# Autodesk Inventor assembly: Gearbox2F
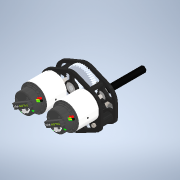
[picture p0: Inventor's stored thumbnail of the model, 180x180]
Saved by Autodesk Inventor 2022 (Build 260153000, 153)
## iProperties
Created: 2022-01-10
Part Number: Gearbox2F
Document SubType Name: Assembly
Designer: merky
Author: merky
## Documents named in this file (7)
- C:\Users\Daniel Marquez\Documents\t3-cad\CAD\2022 Parts\Generic\Gearbox2F.iam
- C:\Users\Daniel Marquez\Documents\t3-cad\CAD\WCP SS_Shrinkwrap.ipt
- C:\Users\Daniel Marquez\Documents\t3-cad\CAD\2022 Parts\Generic\Falcon500.ipt
- C:\Users\Daniel Marquez\Documents\t3-cad\CAD\WCP DS Gearbox\217-2734.ipt
- C:\Users\Daniel Marquez\Documents\t3-cad\CAD\WCP DS Gearbox\217-3422-007 Rev1.ipt
- C:\Users\Daniel Marquez\Documents\t3-cad\CAD\WCP DS Gearbox\217-3422-004 Rev2.ipt
- C:\Users\Daniel Marquez\Documents\t3-cad\CAD\2022 Parts\Generic\9inthundershaft.ipt
## Components (8 placed, 6 different names)
1. WCP SS_Shrinkwrap:1 — Insert:1, Insert:2, Insert:5
2. Falcon500:1 — Insert:2
3. Falcon500:2 — Insert:1
4. 217-2734:1 — Mate:5, Mate:6
5. 217-3422-007 Rev1:1 — Insert:4
6. 217-3422-007 Rev1:2 — Insert:3
7. 217-3422-004 Rev2:1 — Insert:3, Insert:4, Insert:5
8. 9inthundershaft:1 — Mate:5, Mate:6
## Relationships (9: Insert 5, Mate 4)
- Insert:1: WCP SS_Shrinkwrap:1 ↔ Falcon500:2
- Insert:2: WCP SS_Shrinkwrap:1 ↔ Falcon500:1
- [Mate]: 217-2734:1 ↔ 217-3422-004 Rev2:1
- [Mate]: 217-2734:1 ↔ 217-3422-004 Rev2:1
- Insert:3: 217-3422-007 Rev1:2 ↔ 217-3422-004 Rev2:1
- Insert:4: 217-3422-007 Rev1:1 ↔ 217-3422-004 Rev2:1
- Insert:5 (-28.575 mm): WCP SS_Shrinkwrap:1 ↔ 217-3422-004 Rev2:1
- Mate:5: 217-2734:1 ↔ 9inthundershaft:1
- Mate:6: 217-2734:1 ↔ 9inthundershaft:1
## Named parameters: d4_d5 = 0 mm
